# Autodesk Inventor assembly: Arm
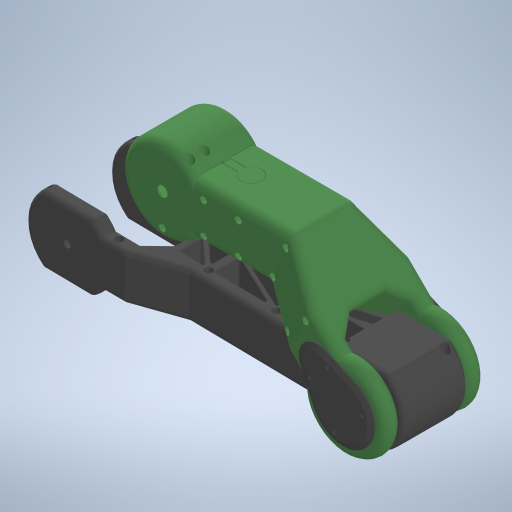
[picture p0: Inventor's stored thumbnail of the model, 512x512]
Saved by Autodesk Inventor 2023 (Build 270158000, 158)
## iProperties
Created: 2024-07-28
Part Number: Arm
Document SubType Name: Assembly
Designer: Swoby
Author: Swoby
## Documents named in this file (7)
- C:\Users\Swoby\OneDrive\Plocha\DUM-E\V0.3\NewArm\Arm.iam
- C:\Users\Swoby\OneDrive\Plocha\DUM-E\V0.3\NewArm\Arm_1L.ipt
- C:\Users\Swoby\OneDrive\Plocha\DUM-E\V0.3\NewArm\Arm_1R.ipt
- C:\Users\Swoby\OneDrive\Plocha\DUM-E\V0.3\NewArm\Arm_1_Cover.ipt
- C:\Users\Swoby\OneDrive\Plocha\DUM-E\V0.3\NewArm\Arm_1Up.ipt
- C:\Users\Swoby\OneDrive\Plocha\DUM-E\V0.3\NewArm\Arm_2D.ipt
- C:\Users\Swoby\OneDrive\Plocha\DUM-E\V0.3\NewArm\Arm_2U.ipt
## Components (7 placed, 6 different names)
1. Arm_1L:1 — Mate:1, Mate:2, Mate:3, Mate:6, Mate:7, Mate:8, Flush:1, Mate:12
2. Arm_1R:1 — Mate:1, Mate:2, Mate:3, Mate:4, Mate:9, Mate:10, Mate:11, Mate:13, Mate:14
3. Arm_1_Cover:1 — Mate:6, Mate:7, Mate:8
4. Arm_1_Cover:2 — Mate:4, Mate:9, Mate:10
5. Arm_1Up:1 — Mate:11, Flush:1, Mate:12
6. Arm_2D:1 — Mate:13, Mate:14, Mate:15, Mate:16, Mate:17
7. Arm_2U:1 — Mate:15, Mate:16, Mate:17
## Relationships (17: Mate 16, Flush 1)
- Mate:1: Arm_1L:1 ↔ Arm_1R:1
- Mate:2: Arm_1L:1 ↔ Arm_1R:1
- Mate:3: Arm_1L:1 ↔ Arm_1R:1
- Mate:4: Arm_1R:1 ↔ Arm_1_Cover:2
- Mate:6: Arm_1L:1 ↔ Arm_1_Cover:1
- Mate:7: Arm_1L:1 ↔ Arm_1_Cover:1
- Mate:8: Arm_1L:1 ↔ Arm_1_Cover:1
- Mate:9: Arm_1R:1 ↔ Arm_1_Cover:2
- Mate:10: Arm_1R:1 ↔ Arm_1_Cover:2
- Mate:11: Arm_1R:1 ↔ Arm_1Up:1
- Flush:1: Arm_1L:1 ↔ Arm_1Up:1
- Mate:12: Arm_1L:1 ↔ Arm_1Up:1
- Mate:13: Arm_1R:1 ↔ Arm_2D:1
- Mate:14: Arm_1R:1 ↔ Arm_2D:1
- Mate:15: Arm_2D:1 ↔ Arm_2U:1
- Mate:16: Arm_2D:1 ↔ Arm_2U:1
- Mate:17: Arm_2D:1 ↔ Arm_2U:1
